# Autodesk Inventor assembly: ensamble_servos
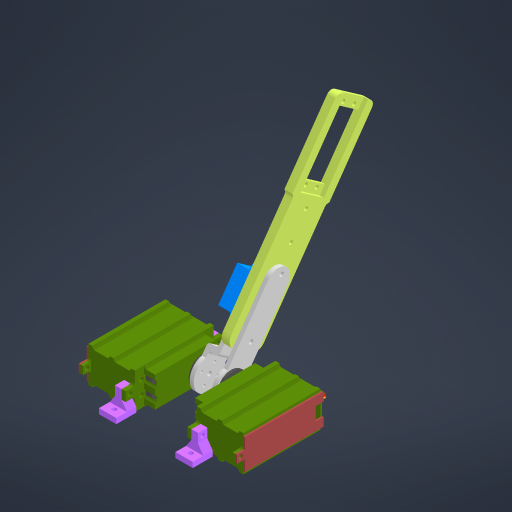
[picture p0: Inventor's stored thumbnail of the model, 512x512]
Saved by Autodesk Inventor 2023.1 (Build 271208000, 208)
## iProperties
Created: 2022-11-07
Part Number: ensamble_servos
Document SubType Name: Assembly
Designer: amtat
Author: amtat
## Documents named in this file (9)
- C:\Users\amtat\OneDrive - uc.cl\UC\Año 5\Sem 2\Capstone\Gripper\ensamble_servos.iam
- C:\Users\amtat\OneDrive - uc.cl\UC\Año 5\Sem 2\Capstone\Gripper\antebrazo.ipt
- C:\Users\amtat\OneDrive - uc.cl\UC\Año 5\Sem 2\Capstone\Gripper\union_servos_1.ipt
- C:\Users\amtat\OneDrive - uc.cl\UC\Año 5\Sem 2\Capstone\Gripper\union_servos_2.ipt
- C:\Users\amtat\OneDrive - uc.cl\UC\Año 5\Sem 2\Capstone\Gripper\TOWER PRO MG-995, ANALOG SERVO v9.iam
- C:\Users\amtat\OneDrive - uc.cl\UC\Año 5\Sem 2\Capstone\Gripper\carcasa_servo.ipt
- C:\Users\amtat\OneDrive - uc.cl\UC\Año 5\Sem 2\Capstone\Gripper\tapa_carcasa.ipt
- C:\Users\amtat\OneDrive - uc.cl\UC\Año 5\Sem 2\Capstone\Gripper\base_servos.ipt
- C:\Users\amtat\OneDrive - uc.cl\UC\Año 5\Sem 2\Capstone\Gripper\carcasa_giroscopio.ipt
## Components (14 placed, 8 different names)
1. antebrazo:1 — Insert:1, Insert:2, Insert:3, Insert:4
2. union_servos_1:1 — Insert:1, Insert:2, Insert:7, Insert:13, Insert:14
3. union_servos_2:1 — Insert:3, Insert:4, Insert:10
4. TOWER PRO MG-995, ANALOG SERVO v9:1 [sub-assembly] — Insert:5, Insert:6, Insert:7
5. carcasa_servo:1 — Insert:5, Insert:6, Flush:1, Flush:2, Flush:3, Mate:1, Insert:16, Mate:4, Insert:17
6. TOWER PRO MG-995, ANALOG SERVO v9:2 [sub-assembly] — Insert:10
7. carcasa_servo:2 — Flush:1, Flush:4, Flush:5, Mate:2, Insert:15, Mate:3, Insert:18
8. tapa_carcasa:1 — Flush:2, Flush:3, Mate:1
9. tapa_carcasa:2 — Flush:4, Flush:5, Mate:2
10. carcasa_giroscopio:1 — Insert:13, Insert:14
11. base_servos:3 — Insert:15, Mate:3
12. base_servos:4 — Insert:16, Mate:4
13. base_servos:5 — Insert:18
14. base_servos:6 — Insert:17
## Relationships (25: Insert 16, Flush 5, Mate 4)
- Insert:1: antebrazo:1 ↔ union_servos_1:1
- Insert:2: antebrazo:1 ↔ union_servos_1:1
- Insert:3: antebrazo:1 ↔ union_servos_2:1
- Insert:4: antebrazo:1 ↔ union_servos_2:1
- Insert:5: TOWER PRO MG-995, ANALOG SERVO v9:1 ↔ carcasa_servo:1
- Insert:6: TOWER PRO MG-995, ANALOG SERVO v9:1 ↔ carcasa_servo:1
- Insert:7: union_servos_1:1 ↔ TOWER PRO MG-995, ANALOG SERVO v9:1
- [Insert]: TOWER PRO MG-995, ANALOG SERVO v9:2 ↔ carcasa_servo:2
- [Insert]: TOWER PRO MG-995, ANALOG SERVO v9:2 ↔ carcasa_servo:2
- Insert:10: union_servos_2:1 ↔ TOWER PRO MG-995, ANALOG SERVO v9:2
- Flush:1: carcasa_servo:1 ↔ carcasa_servo:2
- Flush:2: carcasa_servo:1 ↔ tapa_carcasa:1
- Flush:3: carcasa_servo:1 ↔ tapa_carcasa:1
- Mate:1: carcasa_servo:1 ↔ tapa_carcasa:1
- Flush:4: carcasa_servo:2 ↔ tapa_carcasa:2
- Flush:5: carcasa_servo:2 ↔ tapa_carcasa:2
- Mate:2: carcasa_servo:2 ↔ tapa_carcasa:2
- Insert:13: union_servos_1:1 ↔ carcasa_giroscopio:1
- Insert:14: union_servos_1:1 ↔ carcasa_giroscopio:1
- Insert:15: carcasa_servo:2 ↔ base_servos:3
- Mate:3: carcasa_servo:2 ↔ base_servos:3
- Insert:16: carcasa_servo:1 ↔ base_servos:4
- Mate:4: carcasa_servo:1 ↔ base_servos:4
- Insert:17: carcasa_servo:1 ↔ base_servos:6
- Insert:18: carcasa_servo:2 ↔ base_servos:5
## Named parameters: d11_d8 = 0 mm, d12_d9 = 0 mm
